# Autodesk Inventor assembly: Tamale - V2p0p0
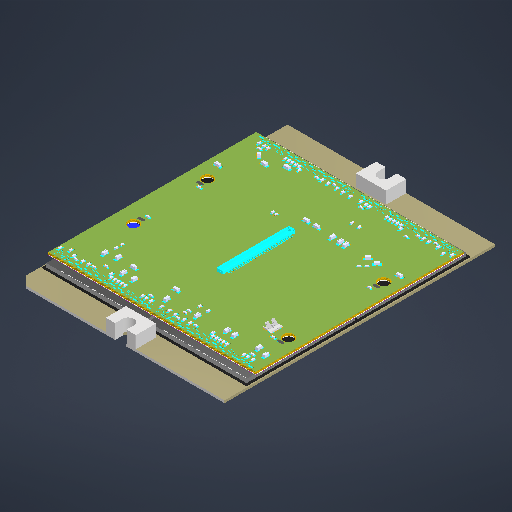
[picture p0: Inventor's stored thumbnail of the model, 512x512]
Saved by Autodesk Inventor 2027 (Build 310192060, 192F)
## iProperties
Created: 2026-07-14
Part Number: Tamale - V2p0p0
Document SubType Name: Assembly
Designer: caleb
Author: caleb
## Documents named in this file (8)
- C:\Users\caleb\Desktop\Shared\Software\Hardware\ETL\modules\Tamale v2.0\Tamale - V2p0p0.iam
- C:\Users\caleb\Desktop\Shared\Software\Hardware\ETL\modules\Tamale v2.0\Baseplate v1.5.1.ipt
- C:\Users\caleb\Desktop\Shared\Software\Hardware\ETL\modules\Tamale v2.0\BBM.iam
- C:\Users\caleb\Desktop\Shared\Software\Hardware\ETL\modules\Tamale v2.0\Sensor Placement Film.ipt
- C:\Users\caleb\Desktop\Shared\Software\Hardware\ETL\modules\Tamale v2.0\PCB Mount Film.ipt
- C:\Users\caleb\Desktop\Shared\Software\Hardware\ETL\modules\Tamale v2.0\module_r50\module_r50.iam
- C:\Users\caleb\Desktop\Shared\Software\Hardware\ETL\modules\Tamale v2.0\Edge Spacer v2p0.ipt
- C:\Users\caleb\Desktop\Shared\Software\Hardware\ETL\modules\Tamale v2.0\Thermal Pad.ipt
## Components (11 placed, 7 different names)
1. Baseplate v1.5.1:1 — Mate:1, Flush:1, Flush:2, Flush:12, Mate:9, Flush:14, Flush:15, Flush:16, Mate:10, Flush:17, Mate:11, Flush:18, Flush:19
2. BBM:1 [sub-assembly] — Flush:3, Flush:4, Flush:5, Mate:3, Flush:7, Mate:4
3. BBM:2 [sub-assembly] — Flush:3, Mate:4, Mate:5, Mate:6, Flush:8, Flush:9, Flush:13
4. Sensor Placement Film:1 — Mate:1, Flush:1, Flush:2, Mate:6, Flush:8, Flush:9
5. BBM:3 [sub-assembly] — Flush:5, Flush:6, Mate:2, Mate:5, Mate:7, Flush:10, Flush:11
6. BBM:4 [sub-assembly] — Flush:4, Flush:6, Mate:2, Mate:3, Flush:7
7. PCB Mount Film:1 — Mate:7, Flush:10, Flush:11, Mate:8
8. module_r50:1 [sub-assembly] — Mate:8, Flush:12, Flush:13
9. Edge Spacer v2p0:1 — Mate:9, Flush:14, Flush:15
10. Edge Spacer v2p0:2 — Flush:16, Mate:10, Flush:17
11. Thermal Pad:1 — Mate:11, Flush:18, Flush:19
## Relationships (30: Flush 19, Mate 11)
- Mate:1: Baseplate v1.5.1:1 ↔ Sensor Placement Film:1
- Flush:1 (4.95 mm): Baseplate v1.5.1:1 ↔ Sensor Placement Film:1
- Flush:2 (0.25 mm): Baseplate v1.5.1:1 ↔ Sensor Placement Film:1
- Flush:3: BBM:1 ↔ BBM:2
- Flush:4: BBM:1 ↔ BBM:4
- Flush:5: BBM:1 ↔ BBM:3
- Flush:6: BBM:3 ↔ BBM:4
- Mate:2 (0.2 mm): BBM:3 ↔ BBM:4
- Mate:3 (0.2 mm): BBM:1 ↔ BBM:4
- Flush:7: BBM:1 ↔ BBM:4
- Mate:4 (0.2 mm): BBM:1 ↔ BBM:2
- Mate:5 (0.2 mm): BBM:2 ↔ BBM:3
- Mate:6: BBM:2 ↔ Sensor Placement Film:1
- Flush:8 (0.5 mm): BBM:2 ↔ Sensor Placement Film:1
- Flush:9 (0.5 mm): BBM:2 ↔ Sensor Placement Film:1
- Mate:7: BBM:3 ↔ PCB Mount Film:1
- Flush:10 (0.5 mm): BBM:3 ↔ PCB Mount Film:1
- Flush:11 (0.5 mm): BBM:3 ↔ PCB Mount Film:1
- Mate:8: PCB Mount Film:1 ↔ module_r50:1
- Flush:12: Baseplate v1.5.1:1 ↔ module_r50:1
- Flush:13 (-0.4235 mm): BBM:2 ↔ module_r50:1
- Mate:9: Baseplate v1.5.1:1 ↔ Edge Spacer v2p0:1
- Flush:14: Baseplate v1.5.1:1 ↔ Edge Spacer v2p0:1
- Flush:15: Baseplate v1.5.1:1 ↔ Edge Spacer v2p0:1
- Flush:16: Baseplate v1.5.1:1 ↔ Edge Spacer v2p0:2
- Mate:10: Baseplate v1.5.1:1 ↔ Edge Spacer v2p0:2
- Flush:17: Baseplate v1.5.1:1 ↔ Edge Spacer v2p0:2
- Mate:11: Baseplate v1.5.1:1 ↔ Thermal Pad:1
- Flush:18 (0.5 mm): Baseplate v1.5.1:1 ↔ Thermal Pad:1
- Flush:19 (-0.5 mm): Baseplate v1.5.1:1 ↔ Thermal Pad:1
